# Autodesk Inventor assembly: HexMotorDirectDriveProtoPlate
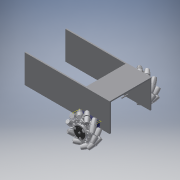
[picture p0: Inventor's stored thumbnail of the model, 180x180]
Saved by Autodesk Inventor 2017 (Build 210142000, 142)
## iProperties
Created: 2017-12-02
Part Number: HexMotorDirectDriveProtoPlate
Document SubType Name: Assembly
Designer: User
Author: User
## Documents named in this file (3)
- C:\Robotics\CAD\2017-18_CAD\Prototypes\HexMotorDirectDriveProtoPlate.iam
- C:\Robotics\CAD\2017-18_CAD\Prototypes\Gen2Plate.ipt
- C:\Robotics\CAD\2017-18_CAD\Prototypes\HexMotorDirectDrive.iam
## Components (3 placed, 2 different names)
1. Gen2Plate:1 — Mate:1, Flush:1, Mate:2, Flush:3, Flush:4, Flush:5
2. HexMotorDirectDrive:1 [sub-assembly] — Mate:2, Flush:3, Flush:5
3. HexMotorDirectDrive:2 [sub-assembly] — Mate:1, Flush:1, Flush:4
## Relationships (6: Flush 4, Mate 2)
- Mate:1: Gen2Plate:1 ↔ HexMotorDirectDrive:2
- Flush:1 (57.15 mm): Gen2Plate:1 ↔ HexMotorDirectDrive:2
- Mate:2: Gen2Plate:1 ↔ HexMotorDirectDrive:1
- Flush:3 (97.79 mm): Gen2Plate:1 ↔ HexMotorDirectDrive:1
- Flush:4 (7.0866 mm): Gen2Plate:1 ↔ HexMotorDirectDrive:2
- Flush:5: Gen2Plate:1 ↔ HexMotorDirectDrive:1
